# Autodesk Inventor assembly: nozz
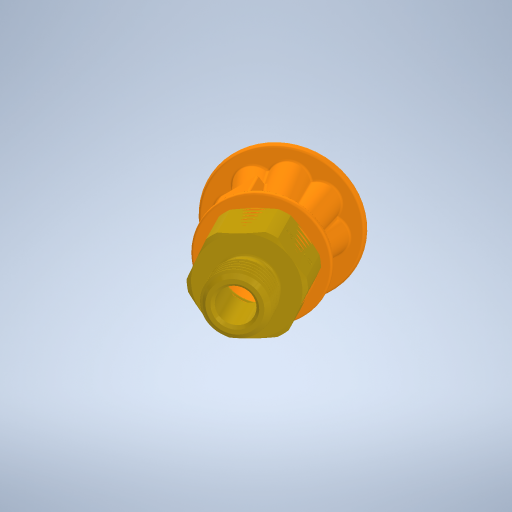
[picture p0: Inventor's stored thumbnail of the model, 512x512]
Saved by Autodesk Inventor 2023 (Build 270158000, 158)
## iProperties
Created: 2023-10-23
Part Number: nozz
Document SubType Name: Assembly
Designer: sigit
Author: sigit
## Documents named in this file (3)
- D:\Kuliah\SEMESTER 7\Robot Semprot\Design\REVISI2\Assembly\nozz.iam
- D:\Kuliah\SEMESTER 7\Robot Semprot\Design\REVISI2\Part\noz.ipt
- D:\Kuliah\SEMESTER 7\Robot Semprot\Design\REVISI2\Part\konektor nz.ipt
## Components (2 placed, 2 different names)
1. noz:1 — Rotational:1
2. konektor nz:1 — Rotational:1
## Relationships (1: RevoluteJoint 1)
- Rotational:1 [RevoluteJoint] (-17 mm): noz:1 ↔ konektor nz:1
